# Autodesk Inventor assembly: DOOROFSHIPCIRCLE
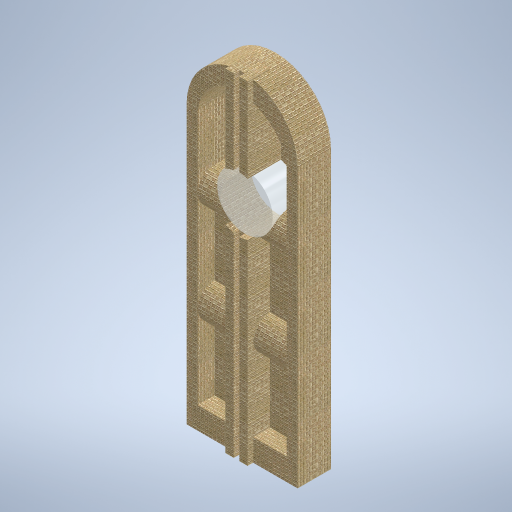
[picture p0: Inventor's stored thumbnail of the model, 512x512]
Saved by Autodesk Inventor 2023 (Build 270158000, 158)
## iProperties
Created: 2023-10-28
Part Number: DOOROFSHIPCIRCLE
Document SubType Name: Assembly
Designer: student
Author: student
## Documents named in this file (3)
- C:\Users\student\Documents\DOOROFSHIPCIRCLE.iam
- C:\Users\student\Documents\circledoor.ipt
- C:\Users\student\Documents\doorship.ipt
## Components (2 placed, 2 different names)
1. circledoor:1 — Rotational:1
2. doorship:1 — Rotational:1
## Relationships (1: RevoluteJoint 1)
- Rotational:1 [RevoluteJoint]: circledoor:1 ↔ doorship:1
